# Autodesk Inventor assembly: structure
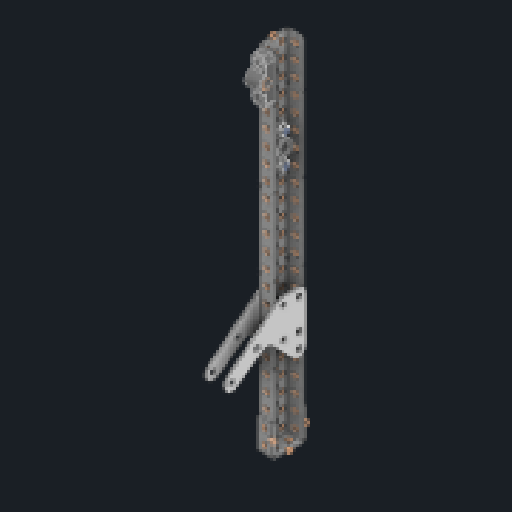
[picture p0: Inventor's stored thumbnail of the model, 512x512]
Saved by Autodesk Inventor 2025 (Build 290162000, 162)
## iProperties
Created: 2024-10-13
Part Number: structure
Document SubType Name: Assembly
Designer: Averey Ku
Author: Averey Ku
## Documents named in this file (10)
- D:\vex_robotics_high_stakes\hardware\cad\bots\high_stakes_v2\tower\structure\vertical.iam
- D:\vex_robotics_high_stakes\hardware\cad\robpros_cad_lib\Structure\C Channel\Aluminum 2x2x2\Alu C 2x2x2x1.ipt
- D:\vex_robotics_high_stakes\hardware\cad\robpros_cad_lib\Structure\C Channel\Aluminum 1x2x1\Alu C 1x2x1x23.ipt
- D:\vex_robotics_high_stakes\hardware\cad\robpros_cad_lib\Motion\Shaft HS\HS Pillow Bearing Block.ipt
- D:\vex_robotics_high_stakes\hardware\cad\bots\high_stakes_v2\tower\structure\custom_parts\triangle_brace_gusset.ipt
- D:\vex_robotics_high_stakes\hardware\cad\robpros_cad_lib\Motion\Shaft HS\HS Bearing Flat.ipt
- D:\vex_robotics_high_stakes\hardware\cad\VEX-CAD-Inventor\Structure\Hardware\Screw Shoulder Robosource\SScrew Shoulder Smooth .500 x .04.ipt
- D:\vex_robotics_high_stakes\hardware\cad\VEX-CAD-Inventor\Structure\Hardware\Screw Shoulder Robosource.ipt
- D:\vex_robotics_high_stakes\hardware\cad\VEX-CAD-Inventor\Structure\Hardware\Nut Nylon\Nut Nylon - White.ipt
- D:\vex_robotics_high_stakes\hardware\cad\VEX-CAD-Inventor\Structure\Hardware\Nut Nylon.ipt
## Components (10 placed, 7 different names)
1. Alu C 2x2x2x1:1 — Mate:2
2. Alu C 1x2x1x23:1 — Insert:4, Mate:5, Insert:6, Mate:7, Insert:7, Mate:8, Insert:10, Mate:11, Insert:11, Insert:12
3. HS Pillow Bearing Block:1 — Insert:4, Mate:5
4. triangle_brace_gusset:1 — Insert:6, Mate:7
5. triangle_brace_gusset:2 — Insert:7, Mate:8
6. HS Bearing Flat:1 — Insert:10, Mate:11
7. SScrew Shoulder Smooth .500 x .04:1 — Insert:12
8. Nut Nylon - White:1
9. SScrew Shoulder Smooth .500 x .04:2 — Insert:11
10. Nut Nylon - White:2
## Relationships (17: Insert 9, Mate 8)
- [Insert]: Alu C 2x2x2x1:1 ↔ Alu C 1x2x1x23:1
- [Mate]: Alu C 2x2x2x1:1 ↔ Alu C 1x2x1x23:1
- Mate:2: Alu C 2x2x2x1:1
- Insert:4: Alu C 1x2x1x23:1 ↔ HS Pillow Bearing Block:1
- Mate:5: Alu C 1x2x1x23:1 ↔ HS Pillow Bearing Block:1
- Insert:6: Alu C 1x2x1x23:1 ↔ triangle_brace_gusset:1
- Mate:7: Alu C 1x2x1x23:1 ↔ triangle_brace_gusset:1
- Insert:7 (12.7 mm): Alu C 1x2x1x23:1 ↔ triangle_brace_gusset:2
- Mate:8: Alu C 1x2x1x23:1 ↔ triangle_brace_gusset:2
- [Mate]: SScrew Shoulder Smooth .500 x .04:1 ↔ Nut Nylon - White:1
- [Insert]: HS Bearing Flat:1 ↔ Nut Nylon - White:1
- [Mate]: SScrew Shoulder Smooth .500 x .04:2 ↔ Nut Nylon - White:2
- [Insert]: HS Bearing Flat:1 ↔ Nut Nylon - White:2
- Insert:10: Alu C 1x2x1x23:1 ↔ HS Bearing Flat:1
- Mate:11: Alu C 1x2x1x23:1 ↔ HS Bearing Flat:1
- Insert:11: Alu C 1x2x1x23:1 ↔ SScrew Shoulder Smooth .500 x .04:2
- Insert:12: Alu C 1x2x1x23:1 ↔ SScrew Shoulder Smooth .500 x .04:1
## Named parameters: d12_d3 = 0 mm, d16_d14 = 0 mm, d15_d12_d3 = 0 mm
